# Autodesk Inventor assembly: Panel Mount Vertical Guide for 4040 - Assembly
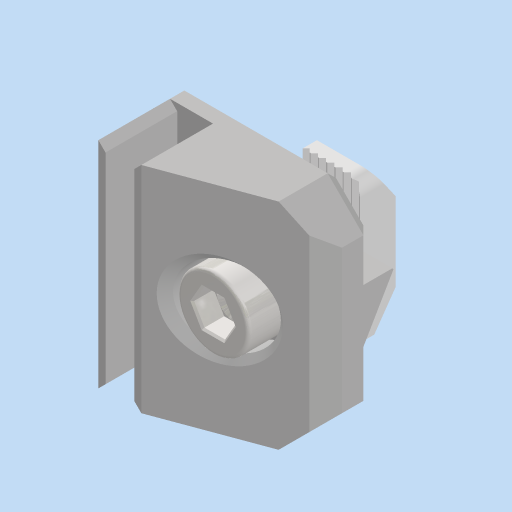
[picture p0: Inventor's stored thumbnail of the model, 512x512]
Saved by Autodesk Inventor 2023.2 (Build 272271000, 271)
## iProperties
Created: 2023-12-04
Part Number: Panel Mount Vertical Guide for 4040 - Assembly
Document SubType Name: Assembly
Designer: Nils Bade
Author: Nils Bade
## Documents named in this file (4)
- C:\Users\nilsb\Documents\Inventor\Projektarbeit-Bade\Enclosure\Panel Mount Vertical Guide for 4040 - Assembly.iam
- C:\Users\nilsb\Documents\Inventor\Projektarbeit-Bade\Enclosure\Panel Mount Vertical Guide for 4040.ipt
- C:\Users\nilsb\Documents\Inventor\Projektarbeit-Bade\Schrauben\Cap Head Screw M6x16.ipt
- C:\Users\nilsb\Documents\Inventor\Projektarbeit-Bade\RatRig_modified\T-NUT - DropIn 4040 SERIES - M6.ipt
## Components (3 placed, 3 different names)
1. Panel Mount Vertical Guide for 4040:1 — Passend:3, Passend:4
2. Cap Head Screw M6x16:1 — Passend:3, Passend:4
3. T-NUT - DROP IN TYPE FOR 40 SERIES - M6:1
## Relationships (5: Mate 4, Angle 1)
- [Mate]: Panel Mount Vertical Guide for 4040:1 ↔ T-NUT - DROP IN TYPE FOR 40 SERIES - M6:1
- [Angle] (0 deg): Panel Mount Vertical Guide for 4040:1 ↔ T-NUT - DROP IN TYPE FOR 40 SERIES - M6:1
- [Mate] (4.5 mm): Panel Mount Vertical Guide for 4040:1 ↔ T-NUT - DROP IN TYPE FOR 40 SERIES - M6:1
- Passend:3 [Mate]: Panel Mount Vertical Guide for 4040:1 ↔ Cap Head Screw M6x16:1
- Passend:4 [Mate]: Panel Mount Vertical Guide for 4040:1 ↔ Cap Head Screw M6x16:1
